# Autodesk Inventor assembly: rail
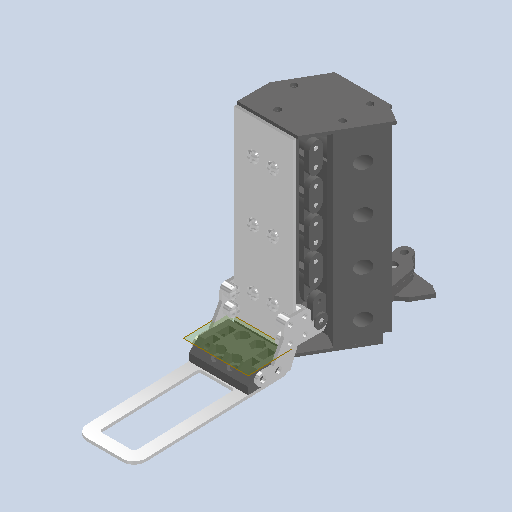
[picture p0: Inventor's stored thumbnail of the model, 512x512]
Saved by Autodesk Inventor 2024.1 (Build 281209000, 209)
## iProperties
Created: 2025-01-17
Part Number: rail
Document SubType Name: Assembly
Designer: hibik
Author: hibik
## Documents named in this file (11)
- C:\Users\hibik\Documents\Robomech\RESCUE\ORCA\hard\fork\right\rail.iam
- C:\Users\hibik\Documents\Robomech\RESCUE\ORCA\hard\fork\right\rail_base.ipt
- C:\Users\hibik\Documents\Robomech\RESCUE\ORCA\hard\fork\right\rail_rail.ipt
- C:\Users\hibik\Documents\Robomech\RESCUE\ORCA\hard\fork\right\rail_cover_upper.ipt
- C:\Users\hibik\Documents\Robomech\RESCUE\ORCA\hard\fork\right\rail_cover_under.ipt
- C:\Users\hibik\Documents\Robomech\RESCUE\ORCA\hard\fork\right\rail_roller.ipt
- C:\Users\hibik\Documents\Robomech\RESCUE\ORCA\hard\fork\right\fork.iam
- C:\Users\hibik\Documents\Robomech\RESCUE\ORCA\hard\fork\right\chain.iam
- C:\Users\hibik\Documents\Robomech\RESCUE\ORCA\hard\std_parts\screw_M3.ipt
- C:\Users\hibik\Documents\Robomech\RESCUE\ORCA\hard\fork\right\screw_lift.iam
- C:\Users\hibik\Documents\Robomech\RESCUE\ORCA\hard\fork\right\rail_backcover.ipt
## Components (15 placed, 10 different names)
1. rail_base:1 — メイト:1, フラッシュ:1, フラッシュ:2, 挿入:1, メイト:6, メイト:7, メイト:8, メイト:9, メイト:10, メイト:11, メイト:13, フラッシュ:7, フラッシュ:8
2. rail_rail:1 — メイト:1, フラッシュ:1, フラッシュ:2, メイト:2, フラッシュ:5, フラッシュ:6, メイト:3, メイト:4, 挿入:2, 挿入:3, 挿入:4, 挿入:5, 挿入:6, 挿入:7, 正接:1, 正接:2
3. rail_cover_upper:1 — メイト:2, メイト:5, メイト:12, フラッシュ:7, フラッシュ:8
4. rail_cover_under:1 — フラッシュ:5, フラッシュ:6, メイト:3
5. rail_roller:1 — 挿入:1
6. fork:1 [sub-assembly] — メイト:4, 正接:1, 正接:2
7. chain:1 [sub-assembly] — メイト:5, メイト:6, メイト:7
8. screw_M3:1 — 挿入:2
9. screw_M3:2 — 挿入:3
10. screw_M3:3 — 挿入:4
11. screw_M3:4 — 挿入:5
12. screw_M3:5 — 挿入:6
13. screw_M3:6 — 挿入:7
14. screw_lift:1 [sub-assembly] — メイト:8, メイト:9, メイト:10
15. rail_backcover:1 — メイト:11, メイト:12, メイト:13
## Relationships (28: Mate 13, Insert 7, Flush 6, Tangent 2)
- メイト:1 [Mate]: rail_base:1 ↔ rail_rail:1
- フラッシュ:1 [Flush]: rail_base:1 ↔ rail_rail:1
- フラッシュ:2 [Flush] (-5 mm): rail_base:1 ↔ rail_rail:1
- メイト:2 [Mate]: rail_rail:1 ↔ rail_cover_upper:1
- フラッシュ:5 [Flush]: rail_rail:1 ↔ rail_cover_under:1
- フラッシュ:6 [Flush]: rail_rail:1 ↔ rail_cover_under:1
- メイト:3 [Mate]: rail_rail:1 ↔ rail_cover_under:1
- 挿入:1 [Insert] (0.25 mm): rail_base:1 ↔ rail_roller:1
- メイト:4 [Mate]: rail_rail:1 ↔ fork:1
- メイト:5 [Mate] (1 mm): rail_cover_upper:1 ↔ chain:1
- メイト:6 [Mate] (1 mm): rail_base:1 ↔ chain:1
- メイト:7 [Mate] (1 mm): rail_base:1 ↔ chain:1
- 挿入:2 [Insert]: rail_rail:1 ↔ screw_M3:1
- 挿入:3 [Insert]: rail_rail:1 ↔ screw_M3:2
- 挿入:4 [Insert]: rail_rail:1 ↔ screw_M3:3
- 挿入:5 [Insert]: rail_rail:1 ↔ screw_M3:4
- 挿入:6 [Insert]: rail_rail:1 ↔ screw_M3:5
- 挿入:7 [Insert]: rail_rail:1 ↔ screw_M3:6
- 正接:1 [Tangent]: rail_rail:1 ↔ fork:1
- 正接:2 [Tangent]: rail_rail:1 ↔ fork:1
- メイト:8 [Mate] (0.2 mm): rail_base:1 ↔ screw_lift:1
- メイト:9 [Mate] (0.1 mm): rail_base:1 ↔ screw_lift:1
- メイト:10 [Mate] (0.1 mm): rail_base:1 ↔ screw_lift:1
- メイト:11 [Mate]: rail_base:1 ↔ rail_backcover:1
- メイト:12 [Mate]: rail_cover_upper:1 ↔ rail_backcover:1
- メイト:13 [Mate]: rail_base:1 ↔ rail_backcover:1
- フラッシュ:7 [Flush]: rail_base:1 ↔ rail_cover_upper:1
- フラッシュ:8 [Flush]: rail_base:1 ↔ rail_cover_upper:1
